# Autodesk Inventor assembly: Assembly1
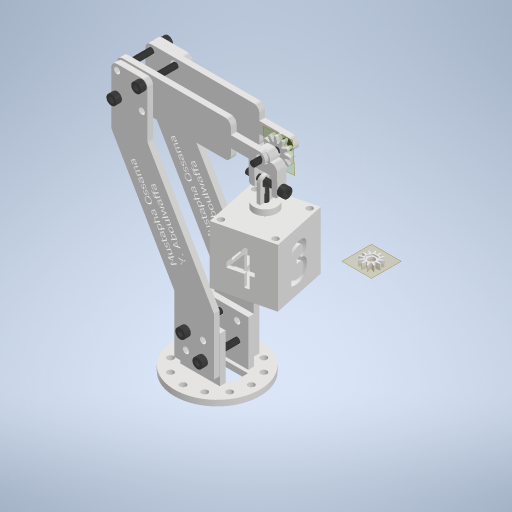
[picture p0: Inventor's stored thumbnail of the model, 512x512]
Saved by Autodesk Inventor 2023 (Build 270158000, 158)
## iProperties
Created: 2023-12-18
Part Number: Assembly1
Document SubType Name: Assembly
Designer: Mustapha
Author: Mustapha
## Documents named in this file (11)
- D:\EDU\Senior 2\Robotics\Activity\Activity New\Assembly1.iam
- D:\EDU\Senior 2\Robotics\Activity\Activity New\Base.ipt
- D:\EDU\Senior 2\Robotics\Activity\Activity New\M5 Hex Screw v2.ipt
- D:\EDU\Senior 2\Robotics\Activity\Activity New\Arm1.ipt
- D:\EDU\Senior 2\Robotics\Activity\Activity New\Arm2.ipt
- D:\EDU\Senior 2\Robotics\Activity\Activity New\J1.ipt
- D:\EDU\Senior 2\Robotics\Activity\Activity New\J2.ipt
- D:\EDU\Senior 2\Robotics\Activity\Activity New\Box.ipt
- D:\EDU\Senior 2\Robotics\Activity\Activity New\BoxLed.ipt
- D:\EDU\Senior 2\Robotics\Activity\Activity New\JointFixer.ipt
- D:\EDU\Senior 2\Robotics\Activity\Activity New\JointFixeSmallr.ipt
## Components (22 placed, 10 different names)
1. Base:1 — Mate:2, Mate:4, Angle:1, Mate:6, Angle:2, Mate:9, Mate:12, Mate:13
2. M5 Hex Screw v2:3 — Mate:2, Mate:5, Mate:7
3. M5 Hex Screw v2:4 — Mate:4, Mate:8
4. Arm1:1 — Mate:5, Angle:1, Mate:6, Mate:7, Mate:8, Mate:16, Mate:17, Mate:18, Mate:19, Mate:21, Mate:22, Angle:4
5. Arm1:2 — Angle:2, Mate:10, Mate:11, Mate:12, Mate:14, Mate:15, Mate:23, Mate:24, Mate:25, Mate:26, Mate:28, Mate:31, Angle:3
6. M5 Hex Screw v2:5 — Mate:9, Mate:10, Mate:11
7. M5 Hex Screw v2:6 — Mate:13, Mate:14, Mate:15
8. M5 Hex Screw v2:7 — Mate:18, Mate:19, Mate:21
9. M5 Hex Screw v2:8 — Mate:16, Mate:17, Mate:20
10. Arm2:1 — Mate:20, Mate:22, Angle:4
11. Arm2:2 — Mate:27, Mate:28, Mate:29, Mate:30, Angle:3
12. M5 Hex Screw v2:9 — Mate:23, Mate:24, Mate:27
13. M5 Hex Screw v2:10 — Mate:25, Mate:26, Mate:31
14. M5 Hex Screw v2:11 — Mate:29, Mate:30, Rotational:1, Cylindrical:1
15. J1:1 — Rotational:1, Mate:32, Mate:33
16. M5 Hex Screw v2:13 — Mate:32, Mate:33, Rotational:2
17. J2:1 — Rotational:2, Rotational:3
18. Box:2 — Mate:36, Flush:1, Flush:2
19. BoxLed:1 — Mate:34, Mate:35, Mate:36, Flush:1, Flush:2
20. M5 Hex Screw v2:14 — Mate:34, Mate:35, Rotational:3
21. JointFixer:1 — Cylindrical:1
22. JointFixeSmallr:1
## Relationships (44: Mate 34, Angle 4, RevoluteJoint 3, Flush 2, CylindricalJoint 1)
- Mate:2: Base:1 ↔ M5 Hex Screw v2:3
- Mate:4: Base:1 ↔ M5 Hex Screw v2:4
- Mate:5: M5 Hex Screw v2:3 ↔ Arm1:1
- Angle:1 (0 deg): Base:1 ↔ Arm1:1
- Mate:6: Base:1 ↔ Arm1:1
- Mate:7: M5 Hex Screw v2:3 ↔ Arm1:1
- Mate:8: M5 Hex Screw v2:4 ↔ Arm1:1
- Angle:2 (0 deg): Base:1 ↔ Arm1:2
- Mate:9: Base:1 ↔ M5 Hex Screw v2:5
- Mate:10: Arm1:2 ↔ M5 Hex Screw v2:5
- Mate:11: Arm1:2 ↔ M5 Hex Screw v2:5
- Mate:12: Base:1 ↔ Arm1:2
- Mate:13: Base:1 ↔ M5 Hex Screw v2:6
- Mate:14: Arm1:2 ↔ M5 Hex Screw v2:6
- Mate:15: Arm1:2 ↔ M5 Hex Screw v2:6
- Mate:16: Arm1:1 ↔ M5 Hex Screw v2:8
- Mate:17: Arm1:1 ↔ M5 Hex Screw v2:8
- Mate:18: Arm1:1 ↔ M5 Hex Screw v2:7
- Mate:19: Arm1:1 ↔ M5 Hex Screw v2:7
- Mate:20: M5 Hex Screw v2:8 ↔ Arm2:1
- Mate:21: Arm1:1 ↔ M5 Hex Screw v2:7
- Mate:22: Arm1:1 ↔ Arm2:1
- Mate:23: Arm1:2 ↔ M5 Hex Screw v2:9
- Mate:24: Arm1:2 ↔ M5 Hex Screw v2:9
- Mate:25: Arm1:2 ↔ M5 Hex Screw v2:10
- Mate:26: Arm1:2 ↔ M5 Hex Screw v2:10
- Mate:27: Arm2:2 ↔ M5 Hex Screw v2:9
- Mate:28: Arm1:2 ↔ Arm2:2
- Mate:29: Arm2:2 ↔ M5 Hex Screw v2:11
- Mate:30 (-6 mm): Arm2:2 ↔ M5 Hex Screw v2:11
- Mate:31: Arm1:2 ↔ M5 Hex Screw v2:10
- Rotational:1 [RevoluteJoint]: M5 Hex Screw v2:11 ↔ J1:1
- Angle:3 (0 deg): Arm1:2 ↔ Arm2:2
- Mate:32: J1:1 ↔ M5 Hex Screw v2:13
- Mate:33: J1:1 ↔ M5 Hex Screw v2:13
- Rotational:2 [RevoluteJoint]: M5 Hex Screw v2:13 ↔ J2:1
- Mate:34: BoxLed:1 ↔ M5 Hex Screw v2:14
- Mate:35: BoxLed:1 ↔ M5 Hex Screw v2:14
- Mate:36: Box:2 ↔ BoxLed:1
- Flush:1: Box:2 ↔ BoxLed:1
- Flush:2: Box:2 ↔ BoxLed:1
- Rotational:3 [RevoluteJoint] (-2 mm): J2:1 ↔ M5 Hex Screw v2:14
- Angle:4 (0 deg): Arm1:1 ↔ Arm2:1
- Cylindrical:1: M5 Hex Screw v2:11 ↔ JointFixer:1
